# Autodesk Inventor assembly: Assembly2
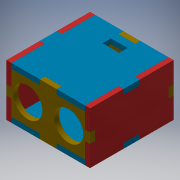
[picture p0: Inventor's stored thumbnail of the model, 180x180]
Saved by Autodesk Inventor 2019 (Build 230136000, 136)
## iProperties
Created: 2020-03-11
Part Number: Assembly2
Document SubType Name: Assembly
Designer: tor16003
Author: tor16003
## Documents named in this file (6)
- E:\Proyecto\Assembly2.iam
- E:\Proyecto\Part5.ipt
- E:\Proyecto\Part8.ipt
- E:\Proyecto\Part6.ipt
- E:\Proyecto\Part7.ipt
- E:\Proyecto\Part9.ipt
## Components (6 placed, 5 different names)
1. Part5:1 — Mate:1, Mate:2, Mate:3, Mate:15, Mate:18, Mate:20
2. Part8:1 — Mate:1, Mate:2, Mate:3, Mate:4, Mate:5, Mate:6, Mate:7, Mate:8, Mate:9, Mate:10, Mate:11, Mate:12, Mate:13
3. Part6:1 — Mate:4, Mate:5, Mate:6
4. Part7:1 — Mate:7, Mate:8, Mate:9, Mate:10, Mate:17, Mate:19, Mate:21
5. Part7:2 — Mate:11, Mate:12, Mate:13, Mate:14, Mate:16
6. Part9:1 — Mate:14, Mate:15, Mate:16, Mate:17, Mate:18, Mate:19, Mate:20, Mate:21
## Relationships (21: Mate 21)
- Mate:1: Part5:1 ↔ Part8:1
- Mate:2: Part5:1 ↔ Part8:1
- Mate:3: Part5:1 ↔ Part8:1
- Mate:4: Part8:1 ↔ Part6:1
- Mate:5: Part8:1 ↔ Part6:1
- Mate:6: Part8:1 ↔ Part6:1
- Mate:7: Part8:1 ↔ Part7:1
- Mate:8: Part8:1 ↔ Part7:1
- Mate:9: Part8:1 ↔ Part7:1
- Mate:10: Part8:1 ↔ Part7:1
- Mate:11: Part8:1 ↔ Part7:2
- Mate:12: Part8:1 ↔ Part7:2
- Mate:13: Part8:1 ↔ Part7:2
- Mate:14: Part7:2 ↔ Part9:1
- Mate:15: Part5:1 ↔ Part9:1
- Mate:16: Part7:2 ↔ Part9:1
- Mate:17: Part7:1 ↔ Part9:1
- Mate:18: Part5:1 ↔ Part9:1
- Mate:19: Part7:1 ↔ Part9:1
- Mate:20: Part5:1 ↔ Part9:1
- Mate:21: Part7:1 ↔ Part9:1
